# Autodesk Inventor assembly: Climb_Assembly
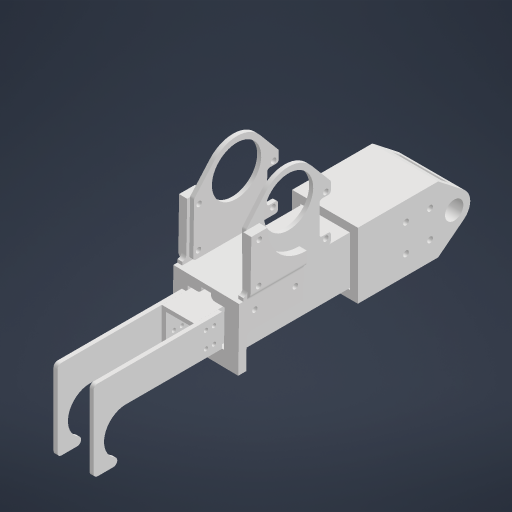
[picture p0: Inventor's stored thumbnail of the model, 512x512]
Saved by Autodesk Inventor 2023 (Build 270158000, 158)
## iProperties
Created: 2024-02-19
Part Number: Climb_Assembly
Document SubType Name: Assembly
Designer: kelle
Author: kelle
## Documents named in this file (8)
- C:\Users\kelle\OneDrive\Documents\Climb_Assembly.iam
- C:\Users\kelle\OneDrive\Documents\CS_Climb_Outer_Tube.ipt
- C:\Users\kelle\OneDrive\Documents\CS_Climb_Outer_Tube_End_Cap.ipt
- C:\Users\kelle\OneDrive\Documents\Outer_Tube_Worm_Connector.ipt
- C:\Users\kelle\OneDrive\Documents\Worm_Gear_Plate_JB.ipt
- C:\Users\kelle\OneDrive\Documents\CS_Climb_Inner_Tube.ipt
- C:\Users\kelle\OneDrive\Documents\CS_Climb_Inner_Tube_End_Cap.ipt
- C:\Users\kelle\OneDrive\Documents\Climb_Hooks_2.ipt
## Components (9 placed, 7 different names)
1. CS_Climb_Outer_Tube:1 — Mate:1, Angle:1, Mate:2, Angle:2, Angle:4, Mate:6
2. CS_Climb_Outer_Tube_End_Cap:1 — Mate:1
3. Outer_Tube_Worm_Connector:1 — Angle:1, Mate:2, Angle:3, Mate:3, Mate:4
4. Worm_Gear_Plate_JB:1 — Angle:2, Angle:3, Mate:3
5. Worm_Gear_Plate_JB:2 — Mate:4
6. CS_Climb_Inner_Tube:1 — Angle:4, Angle:5, Mate:5, Angle:6, Mate:7, Mate:8
7. CS_Climb_Inner_Tube_End_Cap:1 — Angle:5, Mate:5, Mate:6
8. Climb_Hooks_2:1 — Angle:6, Mate:7
9. Climb_Hooks_2:2 — Mate:8
## Relationships (14: Mate 8, Angle 6)
- Mate:1: CS_Climb_Outer_Tube:1 ↔ CS_Climb_Outer_Tube_End_Cap:1
- Angle:1 (0 deg): CS_Climb_Outer_Tube:1 ↔ Outer_Tube_Worm_Connector:1
- Mate:2: CS_Climb_Outer_Tube:1 ↔ Outer_Tube_Worm_Connector:1
- Angle:2 (0 deg): CS_Climb_Outer_Tube:1 ↔ Worm_Gear_Plate_JB:1
- Angle:3 (0 deg): Outer_Tube_Worm_Connector:1 ↔ Worm_Gear_Plate_JB:1
- Mate:3: Outer_Tube_Worm_Connector:1 ↔ Worm_Gear_Plate_JB:1
- Mate:4: Outer_Tube_Worm_Connector:1 ↔ Worm_Gear_Plate_JB:2
- Angle:4 (0 deg): CS_Climb_Outer_Tube:1 ↔ CS_Climb_Inner_Tube:1
- Angle:5 (0 deg): CS_Climb_Inner_Tube:1 ↔ CS_Climb_Inner_Tube_End_Cap:1
- Mate:5: CS_Climb_Inner_Tube:1 ↔ CS_Climb_Inner_Tube_End_Cap:1
- Mate:6: CS_Climb_Outer_Tube:1 ↔ CS_Climb_Inner_Tube_End_Cap:1
- Angle:6 (180 deg): CS_Climb_Inner_Tube:1 ↔ Climb_Hooks_2:1
- Mate:7: CS_Climb_Inner_Tube:1 ↔ Climb_Hooks_2:1
- Mate:8: CS_Climb_Inner_Tube:1 ↔ Climb_Hooks_2:2
